# Autodesk Inventor assembly: element
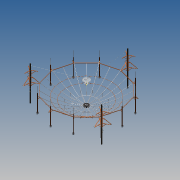
[picture p0: Inventor's stored thumbnail of the model, 180x180]
Saved by Autodesk Inventor 2014 SP1 (Build 180222100, 222)
## iProperties
Created: 2013-12-02
Part Number: element
Document SubType Name: Assembly
Designer: Dave
Author: Dave
## Documents named in this file (27)
- C:\Users\Dave\Desktop\hera-cad\element.iam
- C:\Users\Dave\Desktop\hera-cad\plat.ipt
- C:\Users\Dave\Desktop\hera-cad\hub\hub.iam
- C:\Users\Dave\Desktop\hera-cad\support\poleAssembly.iam
- C:\Users\Dave\Desktop\hera-cad\support\postAssembly.iam
- C:\Users\Dave\Desktop\hera-cad\surface\sparFull.ipt
- C:\Users\Dave\Desktop\hera-cad\support\sparAssembly.iam
- C:\Users\Dave\Desktop\hera-cad\surface\crossAssembly.iam
- C:\Users\Dave\Desktop\hera-cad\surface\sparIntermediate.ipt
- C:\Users\Dave\Desktop\hera-cad\surface\panelA.ipt
- C:\Users\Dave\Desktop\hera-cad\surface\panelB.ipt
- C:\Users\Dave\Desktop\hera-cad\surface\panelC.ipt
- C:\Users\Dave\Desktop\hera-cad\surface\panelD.ipt
- C:\Users\Dave\Desktop\hera-cad\surface\panelE.ipt
- C:\Users\Dave\Desktop\hera-cad\support\rimAssembly.iam
- C:\Users\Dave\Desktop\hera-cad\feed\feedAssembly.iam
- C:\Users\Dave\Desktop\hera-cad\support\furringStrip1.ipt
- C:\Users\Dave\Desktop\hera-cad\support\furringStrip2.ipt
- C:\Users\Dave\Desktop\hera-cad\support\kevlarFeed.ipt
- C:\Users\Dave\Desktop\hera-cad\surface\screenInt.ipt
- C:\Users\Dave\Desktop\hera-cad\surface\ramp.ipt
- C:\Users\Dave\Desktop\hera-cad\surface\panelBdoor.ipt
- C:\Users\Dave\Desktop\hera-cad\jigs\totalStation.ipt
- C:\Users\Dave\Desktop\hera-cad\jigs\vertex.ipt
- C:\Users\Dave\Desktop\hera-cad\support\postStandSupport.iam
- C:\Users\Dave\Desktop\hera-cad\jigs\centering.iam
- C:\Users\Dave\Desktop\hera-cad\jigs\hubjig.iam
## Components (254 placed, 28 different names)
1. plat:1 — Insert:1, Insert:2, Insert:3, Insert:4, Insert:5, Mate:5, Angle:1, Angle:2, Angle:3, Angle:4, Angle:7
2. hub:1 [sub-assembly] — Insert:1, Insert:9, Angle:5, Angle:7, Insert:19, Insert:22, Insert:23, Angle:11, Angle:12, Insert:24, Angle:13
3. feedAssembly:1 [sub-assembly] — Insert:9, Insert:17, Angle:13
4. ramp:1 — Mate:5
5. panelBdoor:1
6. vertex:1 — Insert:19, Insert:20
7. totalStation:1 — Insert:20
8. centeringjig:1 [sub-assembly] — Insert:21
9. hubjig:1 [sub-assembly] — Insert:22
10. panelA:1
11. panelA:2
12. panelA:3
13. panelA:4
14. panelA:5
15. panelA:6
16. panelA:7
17. panelA:8
18. panelA:9
19. panelA:10
20. panelA:11
21. panelA:12
22. panelB:1
23. panelB:2
24. panelB:3
25. panelB:4
26. panelB:5
27. panelB:6
28. panelB:7
29. panelB:8
30. panelB:9
31. panelB:10
32. panelB:11
33. panelB:12
34. panelB:13
35. panelB:14
36. panelB:15
37. panelB:16
38. panelB:17
39. panelB:18
40. panelB:19
41. panelB:20
42. panelB:21
43. panelB:22
44. panelB:23
45. panelC:1
46. panelD:1
47. panelE:1
48. panelC:2
49. panelD:2
50. panelE:2
51. panelC:3
52. panelD:3
53. panelE:3
54. panelC:4
55. panelD:4
56. panelE:4
57. panelC:5
58. panelD:5
59. panelE:5
60. panelC:6
61. panelD:6
62. panelE:6
63. panelC:7
64. panelD:7
65. panelE:7
66. panelC:8
67. panelD:8
68. panelE:8
69. panelC:9
70. panelD:9
71. panelE:9
72. panelC:10
73. panelD:10
74. panelE:10
75. panelC:11
76. panelD:11
77. panelE:11
78. panelC:12
79. panelD:12
80. panelE:12
81. panelC:13
82. panelD:13
83. panelE:13
84. panelC:14
85. panelD:14
86. panelE:14
87. panelC:15
88. panelD:15
89. panelE:15
90. panelC:16
91. panelD:16
92. panelE:16
93. panelC:17
94. panelD:17
95. panelE:17
96. panelC:18
97. panelD:18
98. panelE:18
99. panelC:19
100. panelD:19
101. panelE:19
102. panelC:20
103. panelD:20
104. panelE:20
105. panelC:21
106. panelD:21
107. panelE:21
108. panelC:22
109. panelD:22
110. panelE:22
111. panelC:23
112. panelD:23
113. panelE:23
114. panelC:24
115. panelD:24
116. panelE:24
117. furringStrip2:1
118. furringStrip1:1
119. furringStrip2:2
120. furringStrip1:2
121. furringStrip2:3
122. furringStrip1:3
123. furringStrip2:4
124. furringStrip1:4
125. furringStrip2:5
126. furringStrip1:5
127. furringStrip2:6
128. furringStrip1:6
129. furringStrip2:7
130. furringStrip1:7
131. furringStrip2:8
132. furringStrip1:8
133. furringStrip2:9
134. furringStrip1:9
135. furringStrip2:10
136. furringStrip1:10
137. furringStrip2:11
138. furringStrip1:11
139. furringStrip2:12
140. furringStrip1:12
141. furringStrip2:13
142. furringStrip1:13
143. furringStrip2:14
144. furringStrip1:14
145. furringStrip2:15
146. furringStrip1:15
147. furringStrip2:16
148. furringStrip1:16
149. furringStrip2:17
150. furringStrip1:17
151. furringStrip2:18
152. furringStrip1:18
153. furringStrip2:19
154. furringStrip1:19
155. furringStrip2:20
156. furringStrip1:20
157. furringStrip2:21
158. furringStrip1:21
159. furringStrip2:22
160. furringStrip1:22
161. furringStrip2:23
162. furringStrip1:23
163. furringStrip2:24
164. furringStrip1:24
165. screenInt:1
166. screenInt:2
167. screenInt:3
168. screenInt:4
169. screenInt:5
170. screenInt:6
171. screenInt:7
172. screenInt:8
173. screenInt:9
174. screenInt:10
175. screenInt:11
176. screenInt:12
177. rimAssembly:1 [sub-assembly]
178. rimAssembly:2 [sub-assembly]
179. rimAssembly:3 [sub-assembly]
180. rimAssembly:4 [sub-assembly]
181. rimAssembly:5 [sub-assembly]
182. rimAssembly:6 [sub-assembly]
183. rimAssembly:7 [sub-assembly]
184. rimAssembly:8 [sub-assembly]
185. rimAssembly:9 [sub-assembly]
186. rimAssembly:10 [sub-assembly]
187. rimAssembly:11 [sub-assembly]
188. rimAssembly:12 [sub-assembly]
189. postStandSupport:1 [sub-assembly] — Mate:20, Flush:1, Mate:21
190. postAssembly:1 [sub-assembly] — Insert:5, Angle:4
191. postAssembly:2 [sub-assembly] — Insert:4, Angle:3, Mate:20, Flush:1, Mate:21
192. postAssembly:3 [sub-assembly] — Insert:3, Angle:2
193. postStandSupport:2 [sub-assembly]
194. postAssembly:4 [sub-assembly]
195. postAssembly:5 [sub-assembly]
196. postAssembly:6 [sub-assembly]
197. postStandSupport:3 [sub-assembly]
198. postAssembly:7 [sub-assembly]
199. postAssembly:8 [sub-assembly]
200. postAssembly:9 [sub-assembly]
201. poleAssembly:1 [sub-assembly] — Insert:2, Angle:1, Insert:21
202. poleAssembly:2 [sub-assembly]
203. poleAssembly:3 [sub-assembly]
204. kevlarFeedLine:1 — Insert:17
205. kevlarFeed:2
206. kevlarFeed:3
207. supportSparAssembly:1 [sub-assembly] — Angle:5, Insert:24
208. sparFull:1 — Insert:16, Insert:23, Angle:11
209. crossAssembly:1 [sub-assembly] — Mate:19, Insert:15, Insert:16, Angle:12
210. sparIntermediate:1 — Mate:19, Insert:15
211. sparAssembly:2 [sub-assembly]
212. sparFull:2
213. crossAssembly:2 [sub-assembly]
214. sparIntermediate:2
215. sparAssembly:3 [sub-assembly]
216. sparFull:3
217. crossAssembly:3 [sub-assembly]
218. sparIntermediate:3
219. sparAssembly:4 [sub-assembly]
220. sparFull:4
221. crossAssembly:4 [sub-assembly]
222. sparIntermediate:4
223. sparAssembly:5 [sub-assembly]
224. sparFull:5
225. crossAssembly:5 [sub-assembly]
226. sparIntermediate:5
227. sparAssembly:6 [sub-assembly]
228. sparFull:6
229. crossAssembly:6 [sub-assembly]
230. sparIntermediate:6
231. sparAssembly:7 [sub-assembly]
232. sparFull:7
233. crossAssembly:7 [sub-assembly]
234. sparIntermediate:7
235. sparAssembly:8 [sub-assembly]
236. sparFull:8
237. crossAssembly:8 [sub-assembly]
238. sparIntermediate:8
239. sparAssembly:9 [sub-assembly]
240. sparFull:9
241. crossAssembly:9 [sub-assembly]
242. sparIntermediate:9
243. sparAssembly:10 [sub-assembly]
244. sparFull:10
245. crossAssembly:10 [sub-assembly]
246. sparIntermediate:10
247. sparAssembly:11 [sub-assembly]
248. sparFull:11
249. crossAssembly:11 [sub-assembly]
250. sparIntermediate:11
251. sparAssembly:12 [sub-assembly]
252. sparFull:12
253. crossAssembly:12 [sub-assembly]
254. sparIntermediate:12
## Component patterns: panelA (12 elements), panelB (23 elements), panelC-E (24 elements), furringStrips (24 elements), screen (12 elements), Rim (12 elements), posts (3 elements), poles (3 elements), feedlines (3 elements), (12 elements, first: supportSparAssembly:1 + sparFull:1 + crossAssembly:1 + sparIntermediate:1)
## Relationships (29: Insert 15, Angle 9, Mate 4, Flush 1)
- Insert:1: plat:1 ↔ hub:1
- Insert:2 (-1000 mm): plat:1 ↔ poleAssembly:1
- Insert:3: plat:1 ↔ postAssembly:3
- Insert:4: plat:1 ↔ postAssembly:2
- Insert:5: plat:1 ↔ postAssembly:1
- Insert:9 (4419.6 mm): hub:1 ↔ feedAssembly:1
- Mate:5: plat:1 ↔ ramp:1
- Angle:1 (90 deg): plat:1 ↔ poleAssembly:1
- Angle:2 (180 deg): plat:1 ↔ postAssembly:3
- Angle:3 (210 deg): plat:1 ↔ postAssembly:2
- Angle:4 (150 deg): plat:1 ↔ postAssembly:1
- Angle:5 (180 deg): hub:1 ↔ supportSparAssembly:1
- Mate:19: crossAssembly:1 ↔ sparIntermediate:1
- Insert:15 (-25.4 mm): crossAssembly:1 ↔ sparIntermediate:1
- Angle:7 (180 deg): plat:1 ↔ hub:1
- Insert:16 (2.54 mm): sparFull:1 ↔ crossAssembly:1
- Insert:17: feedAssembly:1 ↔ kevlarFeedLine:1
- Insert:19 (65.1764 mm): hub:1 ↔ vertex:1
- Insert:20 (-1524 mm): vertex:1 ↔ totalStation:1
- Mate:20: postStandSupport:1 ↔ postAssembly:2
- Flush:1: postStandSupport:1 ↔ postAssembly:2
- Mate:21 (1562.1 mm): postStandSupport:1 ↔ postAssembly:2
- Insert:21: centeringjig:1 ↔ poleAssembly:1
- Insert:22 (-76.2 mm): hub:1 ↔ hubjig:1
- Insert:23 (-259.08 mm): hub:1 ↔ sparFull:1
- Angle:11 (180 deg): hub:1 ↔ sparFull:1
- Angle:12 (13.5 deg): hub:1 ↔ crossAssembly:1
- Insert:24 (-25.4 mm): hub:1 ↔ supportSparAssembly:1
- Angle:13 (180 deg): hub:1 ↔ feedAssembly:1
